# Autodesk Inventor assembly: J024 GearMotor
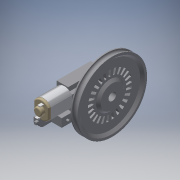
[picture p0: Inventor's stored thumbnail of the model, 180x180]
Saved by Autodesk Inventor 2016 (Build 200138000, 138)
## iProperties
Created: 2016-09-17
Part Number: J024 GearMotor
Document SubType Name: Assembly
Designer: benja
Author: benja
## Documents named in this file (5)
- C:\Users\benja\Google Drive\RIT FIRST club\TigerBug_\CAD\J024 GearMotor.iam
- C:\Users\benja\Google Drive\RIT FIRST club\TigerBug_\CAD\J024 motor.ipt
- C:\Users\benja\Google Drive\RIT FIRST club\TigerBug_\CAD\J024 mount.ipt
- C:\Users\benja\Google Drive\RIT FIRST club\TigerBug_\CAD\j024 output.ipt
- C:\Users\benja\Google Drive\RIT FIRST club\TigerBug_\CAD\wheel.ipt
## Components (4 placed, 4 different names)
1. J024 motor:1 — Mate:1, Mate:2, Tangent:1, Mate:4, Tangent:2
2. J024 mount:1 — Flush:1, Flush:2, Mate:4, Tangent:2
3. j024 output:1 — Flush:2, Mate:3, Mate:5, Mate:6
4. wheel:1 — Mate:3, Mate:5, Mate:6
## Relationships (10: Mate 6, Tangent 2, Flush 2)
- Mate:1: J024 motor:1
- Mate:2: J024 motor:1
- Tangent:1: J024 motor:1
- Flush:1: J024 mount:1
- Flush:2: J024 mount:1 ↔ j024 output:1
- Mate:3: j024 output:1 ↔ wheel:1
- Mate:4: J024 motor:1 ↔ J024 mount:1
- Tangent:2: J024 motor:1 ↔ J024 mount:1
- Mate:5: j024 output:1 ↔ wheel:1
- Mate:6 (0.3 mm): j024 output:1 ↔ wheel:1
